# Autodesk Inventor assembly: 300-009 (TURNBUCKLE ASSEMBLY)
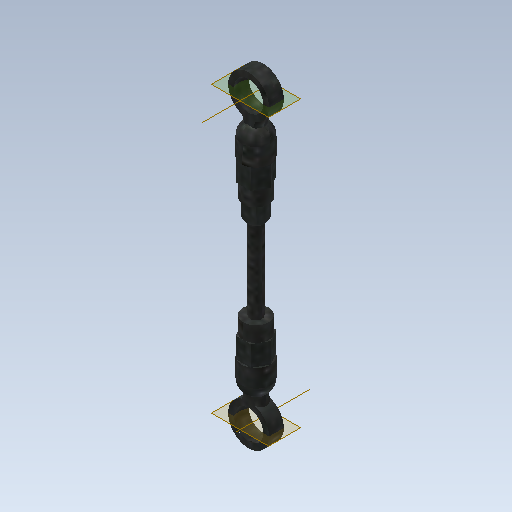
[picture p0: Inventor's stored thumbnail of the model, 512x512]
Saved by Autodesk Inventor 2020 (Build 240168000, 168)
## iProperties
Created: 2015-04-18
Part Number: 300-009 (TURNBUCKLE ASSEMBLY)
Document SubType Name: Assembly
Designer: Station9
Author: Station9
## Documents named in this file (3)
- C:\Users\0x6f736f646f\Downloads\rc-car-16.snapshot.3\300-009 (TURNBUCKLE ASSEMBLY).iam
- C:\Users\0x6f736f646f\Downloads\rc-car-16.snapshot.3\500-001.ipt
- C:\Users\0x6f736f646f\Downloads\rc-car-16.snapshot.3\500-000.ipt
## Components (3 placed, 2 different names)
1. 500-001:1 — Insert:1, Insert:2
2. 500-000:1 — Insert:1
3. 500-000:2 — Insert:2
## Relationships (2: Insert 2)
- Insert:1: 500-001:1 ↔ 500-000:1
- Insert:2 (-6 mm): 500-001:1 ↔ 500-000:2
